# Autodesk Inventor assembly: StopMechanismAssembly_MIR
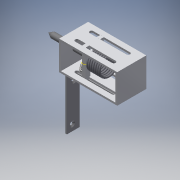
[picture p0: Inventor's stored thumbnail of the model, 180x180]
Saved by Autodesk Inventor 2016 SP1 (Build 200210100, 210)
## iProperties
Created: 2016-02-17
Part Number: StopMechanismAssembly_MIR
Document SubType Name: Assembly
Designer: steele
Mass: 221.776 g
Surface Area: 431.604 cm^2
Volume: 61.0209 cm^3
Density: 3.63442 g/cm^3
Author: steele
## Documents named in this file (9)
- C:\snobotics\CAD-Development\robSteele\SnoBotics2016\2016-02-17-StopMechanism\StopMechanismAssembly_MIR.iam
- C:\snobotics\CAD-Development\robSteele\SnoBotics2016\2016-02-17-StopMechanism\StopMechanismHousing_MIR.ipt
- C:\snobotics\CAD-Development\robSteele\SnoBotics2016\2016-02-17-StopMechanism\outerTubeStopPost_MIR.ipt
- C:\snobotics\CAD-Development\robSteele\SnoBotics2016\2016-02-17-StopMechanism\StopMechanismPushPlate_MIR.ipt
- C:\snobotics\CAD-Development\robSteele\SnoBotics2016\2016-02-17-StopMechanism\StopMechanismAssembly\Design Accelerator\Compress Spring1_MIR.iam
- C:\snobotics\CAD-Development\robSteele\SnoBotics2016\2016-02-17-StopMechanism\StopMechanismAssembly\Design Accelerator\Bolted Connection1.iam
- C:\snobotics\CAD-MfgResources\McMaster-Carr\Bracket\4 Inch\1556A170_MIR.ipt
- C:\snobotics\CAD-Development\robSteele\SnoBotics2016\2016-02-17-StopMechanism\StopMechanismAssembly\Design Accelerator\Bolted Connection3.iam
- C:\snobotics\CAD-Development\robSteele\SnoBotics2016\2016-02-17-StopMechanism\StopMechanismAssembly\Design Accelerator\Bolted Connection4.iam
## Components (8 placed, 6 different names)
1. StopMechanismHousing_MIR:1 — Insert:1, Flush:3, Flush:2, Mate:4
2. outerTubeStopPost_MIR:1 — Insert:1, Insert:2, Mate:10
3. StopMechanismPushPlate_MIR:1 — Insert:2, Flush:1, Mate:1, Mate:9
4. Compress Spring1_MIR:1 [sub-assembly] — Flush:1, Mate:1
5. Bolted Connection:1 [sub-assembly] — Mate:10, Mate:9
6. 1556A170_MIR:1 — Flush:3, Flush:2, Mate:4, Mate:6, Mate:5, Mate:8, Mate:7
7. Bolted Connection:2 [sub-assembly] — Mate:6, Mate:5
8. Bolted Connection:3 [sub-assembly] — Mate:8, Mate:7
## Relationships (13: Mate 9, Insert 2, Flush 2)
- Insert:1 (-30.48 mm): StopMechanismHousing_MIR:1 ↔ outerTubeStopPost_MIR:1
- Insert:2: outerTubeStopPost_MIR:1 ↔ StopMechanismPushPlate_MIR:1
- Flush:1 [Mate]: StopMechanismPushPlate_MIR:1 ↔ Compress Spring1_MIR:1
- Mate:1: StopMechanismPushPlate_MIR:1 ↔ Compress Spring1_MIR:1
- Mate:10: outerTubeStopPost_MIR:1 ↔ Bolted Connection:1
- Mate:9: StopMechanismPushPlate_MIR:1 ↔ Bolted Connection:1
- Flush:3 (-14.2875 mm): StopMechanismHousing_MIR:1 ↔ 1556A170_MIR:1
- Flush:2 (-3.683 mm): StopMechanismHousing_MIR:1 ↔ 1556A170_MIR:1
- Mate:4: StopMechanismHousing_MIR:1 ↔ 1556A170_MIR:1
- Mate:6: 1556A170_MIR:1 ↔ Bolted Connection:2
- Mate:5: 1556A170_MIR:1 ↔ Bolted Connection:2
- Mate:8: 1556A170_MIR:1 ↔ Bolted Connection:3
- Mate:7: 1556A170_MIR:1 ↔ Bolted Connection:3
